# Autodesk Inventor assembly: finger middle
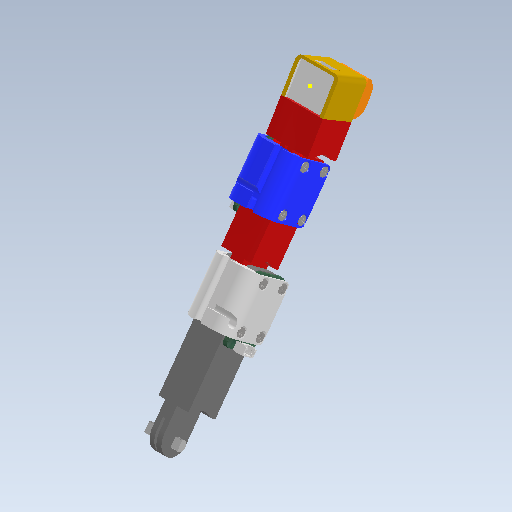
[picture p0: Inventor's stored thumbnail of the model, 512x512]
Saved by Autodesk Inventor 2020 (Build 240168000, 168)
## iProperties
Created: 2020-01-20
Part Number: finger middle
Document SubType Name: Assembly
Designer: sami_
Author: sami_
## Documents named in this file (4)
- C:\Users\sami_\Documents\V1.6\Workgroups\NotInProject\MIDDLE\finger MIDDLE.iam
- C:\Users\sami_\Documents\V1.6\Workgroups\NotInProject\MIDDLE\Fingertip assembly final.iam
- C:\Users\sami_\Documents\V1.6\MiddleL1.iam
- C:\Users\sami_\Documents\V1.6\MiddleL2.iam
## Components (3 placed, 3 different names)
1. Fingertip assembly final:1 [sub-assembly]
2. MiddleL1:1 [sub-assembly]
3. MiddleL2:1 [sub-assembly]
## Relationships (3: RevoluteJoint 2, Mate 1)
- [RevoluteJoint]: MiddleL1:1 ↔ MiddleL2:1
- [Mate]: MiddleL1:1 ↔ MiddleL2:1
- [RevoluteJoint] (0.8 mm): Fingertip assembly final:1 ↔ MiddleL2:1
